# Autodesk Inventor assembly: 25mm Stroke Pneumatic Cylinder
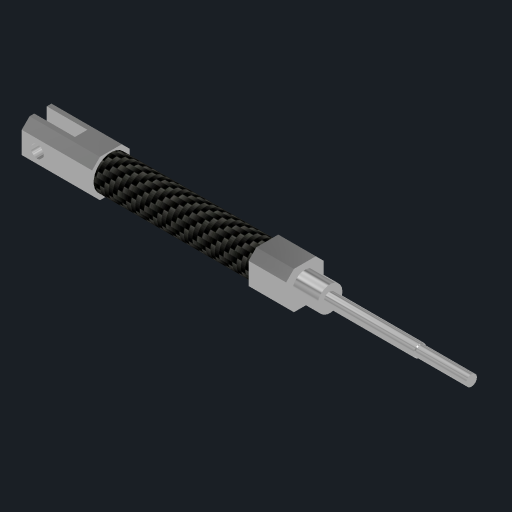
[picture p0: Inventor's stored thumbnail of the model, 512x512]
Saved by Autodesk Inventor 2024.2 (Build 282272000, 272)
## iProperties
Created: 2024-01-31
Part Number: 25mm Stroke Pneumatic Cylinder
Document SubType Name: Assembly
Designer: reima
Sending System: Autodesk Translation Framework v12.14.0.127
Preprocessor: ST-DEVELOPER v20
Title: 25mm Stroke Pneumatic Cylinder v1.step
## Documents named in this file (3)
- O:\cad\61002g-cad\VEX parts\Motion\Pneumatics\25mm Stroke Pneumatic Cylinder v1.iam
- O:\cad\61002g-cad\VEX parts\Motion\Pneumatics\Component1.ipt
- O:\cad\61002g-cad\VEX parts\Motion\Pneumatics\Component2.ipt
## Components (2 placed, 2 different names)
1. Component1:1 — Mate:1, Mate:2
2. Component2:1 — Mate:1, Mate:2
## Relationships (2: Mate 2)
- Mate:1: Component1:1 ↔ Component2:1
- Mate:2: Component1:1 ↔ Component2:1
